# Autodesk Inventor assembly: 12V JGY370-D7 DC Gearmotor
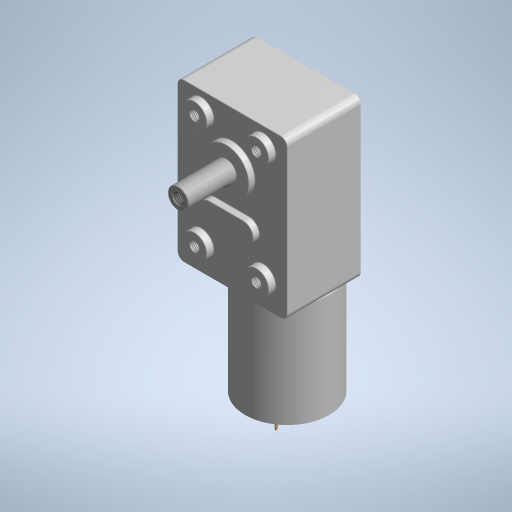
[picture p0: Inventor's stored thumbnail of the model, 512x512]
Saved by Autodesk Inventor 2023 (Build 270158000, 158)
## iProperties
Created: 2022-04-22
Part Number: 12V JGY370-D7 DC Gearmotor
Document SubType Name: Assembly
Designer: Ronan
Sending System: Autodesk Translation Framework v10.14.0.1471
Preprocessor: ST-DEVELOPER v18.1
Title: D:/Documents/_Personal Projects/Electronic Stuff/12V JGY370-D7 DC Gearmotor.step
## Documents named in this file (4)
- D:\Libraries\Documents\2023-FYP\Inventor\JGY-37012V JGY370-D7 DC Gearmotor.iam
- D:\Libraries\Documents\2023-FYP\Inventor\JGY-370Gearbox.ipt
- D:\Libraries\Documents\2023-FYP\Inventor\JGY-370Output Shaft.ipt
- D:\Libraries\Documents\2023-FYP\Inventor\JGY-37012V DC Motor.ipt
## Components (3 placed, 3 different names)
1. Gearbox:1 — Rotational:1, Mate:1, Mate:2, Mate:3
2. Output Shaft:1 — Rotational:1
3. 12V DC Motor:1 — Mate:1, Mate:2, Mate:3
## Relationships (4: Mate 3, RevoluteJoint 1)
- Rotational:1 [RevoluteJoint] (3 mm): Gearbox:1 ↔ Output Shaft:1
- Mate:1 (-8.8 mm): Gearbox:1 ↔ 12V DC Motor:1
- Mate:2 (-13.7 mm): Gearbox:1 ↔ 12V DC Motor:1
- Mate:3: Gearbox:1 ↔ 12V DC Motor:1
